# Autodesk Inventor assembly: Assembly_Cube_Template_rotational_filtermount_v3
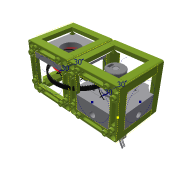
[picture p0: Inventor's stored thumbnail of the model, 180x180]
Saved by Autodesk Inventor 2022 (Build 260153000, 153)
## iProperties
Created: 2020-11-11
Part Number: Assembly_Cube_Template_rotational_filtermount_v3
Document SubType Name: Assembly
Designer: marsikovabarbora
Author: marsikovabarbora
## Documents named in this file (10)
- C:\Users\diederichbenedict\Dropbox\Dokumente\Promotion\PROJECTS\UC2\02_CAD\INVENTOR\uc2_v3\Assembly_Cube_Template_rotational_filtermount_v3.iam
- C:\Users\diederichbenedict\Dropbox\Dokumente\Promotion\PROJECTS\UC2\02_CAD\INVENTOR\uc2_v3\Assembly_Cube_empty_IM_v3.iam
- C:\Users\diederichbenedict\Dropbox\Dokumente\Promotion\PROJECTS\UC2\02_CAD\INVENTOR\uc2_v3\20_Cube_Insert_rotational_filtermount_v3.iam.ipt
- C:\Users\diederichbenedict\Dropbox\Dokumente\Promotion\PROJECTS\UC2\02_CAD\INVENTOR\uc2_v3\20_Cube_Insert_rotational_filtermount_v3.ipt
- C:\Users\diederichbenedict\Dropbox\Dokumente\Promotion\PROJECTS\UC2\02_CAD\INVENTOR\uc2_v3\00_Ballbearing_3x8mm.ipt
- C:\Users\diederichbenedict\Dropbox\Dokumente\Promotion\PROJECTS\UC2\02_CAD\INVENTOR\uc2_v3\00_GT2_TimingBelt_flexible_Modular_xytable_large_89tooth.ipt
- C:\Users\diederichbenedict\Dropbox\Dokumente\Promotion\PROJECTS\UC2\02_CAD\INVENTOR\uc2_v3\30_Cube_Z_Focus_MGN_NEMA_Motorsupport_centered.ipt
- C:\Users\diederichbenedict\Dropbox\Dokumente\Promotion\PROJECTS\UC2\02_CAD\INVENTOR\uc2_v3\00_NEMA11.ipt
- C:\Users\diederichbenedict\Dropbox\Dokumente\Promotion\PROJECTS\UC2\02_CAD\INVENTOR\uc2_v3\00_Gear_Pulley_GT2_nut.ipt
- 20_Cube_Insert_rotational_filtermount_v3.iam
## Components (11 placed, 8 different names)
1. 20_Cube_Insert_rotational_filtermount_v3.iam:1 — Fluchtend:1, Fluchtend:2, Fluchtend:3, Einfügen:1, Einfügen:2, Passend:1, Passend:2, Einfügen:3, Passend:3, Winkel:1
2. 20_Cube_Insert_rotational_filtermount_v3:1 — Fluchtend:1, Fluchtend:2, Einfügen:3
3. 00_Ballbearing_3x8mm:1 — Fluchtend:3
4. 00_Ballbearing_3x8mm:2 — Einfügen:1
5. 00_Ballbearing_3x8mm:3 — Einfügen:2
6. 30_Cube_Z_Focus_MGN_NEMA_Motorsupport_centered:1 — Passend:4, Fluchtend:4, Passend:5, Fluchtend:7
7. 00_NEMA11:1 — Fluchtend:5, Fluchtend:6, Fluchtend:7, Einfügen:4
8. 00_GT2_TimingBelt_flexible_Modular_xytable_large_89tooth:1 — Winkel:1
9. 00_Gear_Pulley_GT2_nut:1 — Einfügen:4
10. Assembly_Cube_empty_IM_v3:2 [sub-assembly] — Passend:1, Passend:2, Passend:3
11. Assembly_Cube_empty_IM_v3:3 [sub-assembly] — Passend:4, Fluchtend:4, Fluchtend:5, Fluchtend:6, Passend:5
## Component patterns: (2 elements, first: Assembly_Cube_empty_IM_v3:2)
## Relationships (17: Flush 7, Mate 5, Insert 4, Angle 1)
- Fluchtend:1 [Flush]: 20_Cube_Insert_rotational_filtermount_v3.iam:1 ↔ 20_Cube_Insert_rotational_filtermount_v3:1
- Fluchtend:2 [Flush]: 20_Cube_Insert_rotational_filtermount_v3.iam:1 ↔ 20_Cube_Insert_rotational_filtermount_v3:1
- Fluchtend:3 [Flush]: 20_Cube_Insert_rotational_filtermount_v3.iam:1 ↔ 00_Ballbearing_3x8mm:1
- Einfügen:1 [Insert]: 20_Cube_Insert_rotational_filtermount_v3.iam:1 ↔ 00_Ballbearing_3x8mm:2
- Einfügen:2 [Insert]: 20_Cube_Insert_rotational_filtermount_v3.iam:1 ↔ 00_Ballbearing_3x8mm:3
- Passend:1 [Mate]: 20_Cube_Insert_rotational_filtermount_v3.iam:1 ↔ Assembly_Cube_empty_IM_v3:2
- Passend:2 [Mate]: 20_Cube_Insert_rotational_filtermount_v3.iam:1 ↔ Assembly_Cube_empty_IM_v3:2
- Einfügen:3 [Insert]: 20_Cube_Insert_rotational_filtermount_v3.iam:1 ↔ 20_Cube_Insert_rotational_filtermount_v3:1
- Passend:3 [Mate]: 20_Cube_Insert_rotational_filtermount_v3.iam:1 ↔ Assembly_Cube_empty_IM_v3:2
- Passend:4 [Mate]: 30_Cube_Z_Focus_MGN_NEMA_Motorsupport_centered:1 ↔ Assembly_Cube_empty_IM_v3:3
- Fluchtend:4 [Flush]: 30_Cube_Z_Focus_MGN_NEMA_Motorsupport_centered:1 ↔ Assembly_Cube_empty_IM_v3:3
- Fluchtend:5 [Flush]: 00_NEMA11:1 ↔ Assembly_Cube_empty_IM_v3:3
- Fluchtend:6 [Flush]: 00_NEMA11:1 ↔ Assembly_Cube_empty_IM_v3:3
- Passend:5 [Mate]: 30_Cube_Z_Focus_MGN_NEMA_Motorsupport_centered:1 ↔ Assembly_Cube_empty_IM_v3:3
- Fluchtend:7 [Flush]: 30_Cube_Z_Focus_MGN_NEMA_Motorsupport_centered:1 ↔ 00_NEMA11:1
- Winkel:1 [Angle] (180 deg): 20_Cube_Insert_rotational_filtermount_v3.iam:1 ↔ 00_GT2_TimingBelt_flexible_Modular_xytable_large_89tooth:1
- Einfügen:4 [Insert]: 00_NEMA11:1 ↔ 00_Gear_Pulley_GT2_nut:1
